# Autodesk Inventor assembly: Chessboard Hardware 2 Model
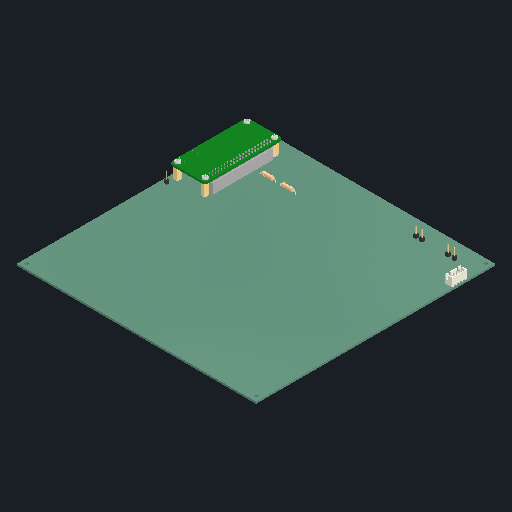
[picture p0: Inventor's stored thumbnail of the model, 512x512]
Saved by Autodesk Inventor 2026 (Build 300175000, 175)
## iProperties
Created: 2025-04-15
Part Number: Chessboard Hardware 2 Model
Document SubType Name: Assembly
Designer: ckyiu
Author: ckyiu
## iProperties of the stored document R_Axial_DIN0309_L90mm_D32mm_P1270mm_Horizontal.ipt
Created: 2025-04-15
Part Number: R_Axial_DIN0309_L90mm_D32mm_P1270mm_Horizontal
Material: Generic
Document SubType Name: Modeling
Designer: ckyiu
Density: 1 g/cm^3
Appearance: Default
Author: ckyiu
## iProperties of the stored document Chessboard-Hardware-2_PCB.ipt
Created: 2025-04-15
Part Number: Chessboard-Hardware-2_PCB
Material: Generic
Document SubType Name: Modeling
Designer: ckyiu
Density: 1 g/cm^3
Appearance: Default
Author: ckyiu
## iProperties of the stored document PinHeader_1x01_P2.54mm_Vertical.iam
Created: 2025-04-15
Part Number: PinHeader_1x01_P2.54mm_Vertical
Document SubType Name: Assembly
Designer: ckyiu
Author: ckyiu
## iProperties of the stored document R_Axial_DIN0309_L9.0mm_D3.2mm_P12.70mm_Horizontal.iam
Created: 2025-04-15
Part Number: R_Axial_DIN0309_L9.0mm_D3.2mm_P12.70mm_Horizontal
Document SubType Name: Assembly
Designer: ckyiu
Author: ckyiu
## iProperties of the stored document Raspberry Pi Zero WH socketed THT facedown mounting holes v5.iam
Created: 2025-04-15
Part Number: Raspberry Pi Zero WH socketed THT facedown mounting holes v5
Document SubType Name: Assembly
Designer: ckyiu
Author: ckyiu
## iProperties of the stored document JST_XH_B4B-XH-A_1x04_P2.50mm_Vertical.iam
Created: 2025-04-15
Part Number: JST_XH_B4B-XH-A_1x04_P2.50mm_Vertical
Document SubType Name: Assembly
Designer: ckyiu
Author: ckyiu
## iProperties of the stored document PinHeader_1x01_P254mm_Vertical.ipt
Created: 2025-04-15
Part Number: PinHeader_1x01_P254mm_Vertical
Material: Generic
Document SubType Name: Modeling
Designer: ckyiu
Density: 1 g/cm^3
Appearance: Default
Author: ckyiu
## iProperties of the stored document Chessboard Hardware 2 Model.iam
Company: Kicad
Created: 2025-04-14
Part Number: Chessboard Hardware 2 Model
Description: KiCad electronic assembly
Document SubType Name: Assembly
Designer: ckyiu
Authority: Unknown
Sending System: KiCad to STEP converter
Preprocessor: Open CASCADE STEP processor 7.8
Title: Chessboard-Hardware-2.step
Author: Pcbnew
## iProperties of the stored document JST_B4B_XH_A.ipt
Created: 2025-04-15
Part Number: JST_B4B_XH_A
Material: Generic
Document SubType Name: Modeling
Designer: ckyiu
Density: 1 g/cm^3
Appearance: Default
Author: ckyiu
## iProperties of the stored document Raspberry Pi Zero WH socketed THT facedown mounting holes v4.ipt
Created: 2025-04-15
Part Number: Raspberry Pi Zero WH socketed THT facedown mounting holes v4
Material: Generic
Document SubType Name: Modeling
Designer: ckyiu
Density: 1 g/cm^3
Appearance: Default
Author: ckyiu
## Documents named in this file (13)
- F:\Chessboard-Design\Assemblies\PCBs\Chessboard Hardware 2 Model.iam
- **F:\Chessboard-Design\Assemblies\PCBs\Chessboard Hardware 2 Model.iam*LocalDocs*xAaaaqjdaAaaaaaaaAaaaq2yr5a*Chessboard Hardware 2 Model.iam
- **C:\Users\ckyiu\Documents\Projects\Chessboard-Design\Assemblies\PCBs\Chessboard Hardware 2 Model.iam*LocalDocs*xAaaaaydaAaaaaaaaAaaaqapuUc*R_Axial_DIN0309_L90mm_D32mm_P1270mm_Horizontal.ipt
- **C:\Users\ckyiu\Documents\Projects\Chessboard-Design\Assemblies\PCBs\Chessboard Hardware 2 Model.iam*LocalDocs*xAaaaafcaAaaaaaaaAaaaav5bKe*Chessboard-Hardware-2_PCB.ipt
- **C:\Users\ckyiu\Documents\Projects\Chessboard-Design\Assemblies\PCBs\Chessboard Hardware 2 Model.iam*LocalDocs*xAaaaaecaAaaaaaaaAaaaqpubQd*PinHeader_1x01_P2.54mm_Vertical.iam
- **C:\Users\ckyiu\Documents\Projects\Chessboard-Design\Assemblies\PCBs\Chessboard Hardware 2 Model.iam*LocalDocs*xAaaaqkcaAaaaaaaaAaaaaruiCe*PinHeader_1x01_P254mm_Vertical.ipt
- **C:\Users\ckyiu\Documents\Projects\Chessboard-Design\Assemblies\PCBs\Chessboard Hardware 2 Model.iam*LocalDocs*xAaaaatdaAaaaaaaaAaaaanhlOh*R_Axial_DIN0309_L9.0mm_D3.2mm_P12.70mm_Horizontal.iam
- **C:\Users\ckyiu\Documents\Projects\Chessboard-Design\Assemblies\PCBs\Chessboard Hardware 2 Model.iam*LocalDocs*xAaaaazbaAaaaaaaaAaaaamjxSe*Raspberry Pi Zero WH socketed THT facedown mounting holes v5.iam
- **C:\Users\ckyiu\Documents\Projects\Chessboard-Design\Assemblies\PCBs\Chessboard Hardware 2 Model.iam*LocalDocs*xAaaaqycaAaaaaaaaAaaaah2tZc*Raspberry Pi Zero WH socketed THT facedown mounting holes v4.ipt
- **C:\Users\ckyiu\Documents\Projects\Chessboard-Design\Assemblies\PCBs\Chessboard Hardware 2 Model.iam*LocalDocs*xAaaaazaaAaaaaaaaAaaaarowPd*JST_XH_B4B-XH-A_1x04_P2.50mm_Vertical.iam
- **C:\Users\ckyiu\Documents\Projects\Chessboard-Design\Assemblies\PCBs\Chessboard Hardware 2 Model.iam*LocalDocs*xAaaaqxdaAaaaaaaaAaaaqklxJh*JST_B4B_XH_A.ipt
- **C:\Users\ckyiu\Documents\Projects\Chessboard-Design\Assemblies\PCBs\Chessboard Hardware 2 Model.iam*LocalDocs*xAaaaqjdaAaaaaaaaAaaaq2yr5a*Chessboard Hardware 2 Model.iam
- F:\Chessboard-Design\Assemblies\PCBs\Chessboard Hardware 2 Model.step
## Components (1 placed, 1 different names)
1. Chessboard Hardware 2 Model:1 [sub-assembly] — Mate:1, Mate:2, Mate:3
## Relationships (3: Mate 3)
- Mate:1 (-100 mm): Chessboard Hardware 2 Model:1
- Mate:2 (-100 mm): Chessboard Hardware 2 Model:1
- Mate:3: Chessboard Hardware 2 Model:1
